# Autodesk Inventor assembly: BBM Staging Plate Assembly
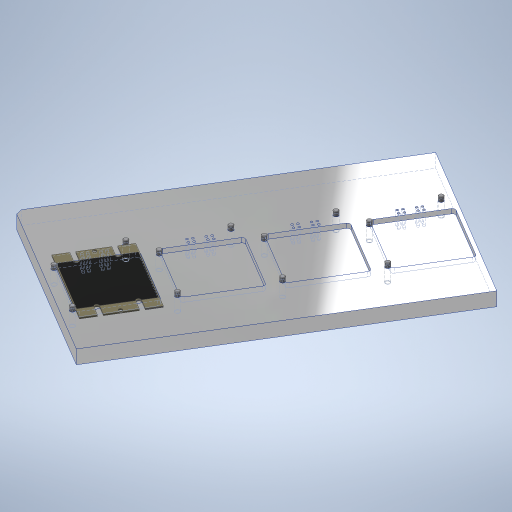
[picture p0: Inventor's stored thumbnail of the model, 512x512]
Saved by Autodesk Inventor 2023 (Build 270158000, 158)
## iProperties
Created: 2021-01-11
Part Number: BBM Staging Plate Assembly
Document SubType Name: Assembly
Designer: caleb
Author: caleb
## Documents named in this file (5)
- C:\Users\Caleb\Desktop\nebraska-silicon-lab\Hardware\ETL\Module Assembly\Baseplate Staging Plate - V2\Baseplate Staging Plate Assembly - V2.iam
- C:\Users\Caleb\Desktop\nebraska-silicon-lab\Hardware\ETL\Module Assembly\Baseplate Staging Plate - V2\Baseplate Staging Plate - V2.ipt
- C:\Users\Caleb\Desktop\nebraska-silicon-lab\Hardware\ETL\Module Assembly\Baseplate Staging Plate - V2\98381A304_Dowel Pin.ipt
- C:\Users\Caleb\Desktop\nebraska-silicon-lab\Hardware\ETL\modules\tamale v1.4\Coverplate Film.ipt
- C:\Users\Caleb\Desktop\nebraska-silicon-lab\Hardware\ETL\modules\tamale v1.4\Baseplate v1.4.ipt
## Components (15 placed, 4 different names)
1. Baseplate Staging Plate - V2:1 — Insert:1, Insert:2, Insert:3, Insert:4, Insert:5, Insert:6, Insert:7, Insert:8, Insert:9, Insert:10, Insert:11, Insert:12, Mate:6, Angle:1
2. 98381A304_Dowel Pin:1 — Insert:3, Tangent:1
3. 98381A304_Dowel Pin:2 — Insert:1, Tangent:2
4. 98381A304_Dowel Pin:3 — Insert:2
5. 98381A304_Dowel Pin:4 — Insert:4
6. 98381A304_Dowel Pin:5 — Insert:5
7. 98381A304_Dowel Pin:6 — Insert:6
8. 98381A304_Dowel Pin:7 — Insert:7
9. 98381A304_Dowel Pin:8 — Insert:8
10. 98381A304_Dowel Pin:9 — Insert:9
11. 98381A304_Dowel Pin:10 — Insert:10
12. 98381A304_Dowel Pin:11 — Insert:11
13. 98381A304_Dowel Pin:12 — Insert:12
14. Coverplate Film:1 — Flush:1, Flush:2
15. Baseplate v1.4:1 — Mate:6, Flush:1, Flush:2, Angle:1, Tangent:1, Tangent:2
## Relationships (19: Insert 12, Mate 2, Flush 2, Tangent 2, Angle 1)
- Insert:1: Baseplate Staging Plate - V2:1 ↔ 98381A304_Dowel Pin:2
- Insert:2: Baseplate Staging Plate - V2:1 ↔ 98381A304_Dowel Pin:3
- Insert:3: Baseplate Staging Plate - V2:1 ↔ 98381A304_Dowel Pin:1
- Insert:4: Baseplate Staging Plate - V2:1 ↔ 98381A304_Dowel Pin:4
- Insert:5: Baseplate Staging Plate - V2:1 ↔ 98381A304_Dowel Pin:5
- Insert:6: Baseplate Staging Plate - V2:1 ↔ 98381A304_Dowel Pin:6
- Insert:7: Baseplate Staging Plate - V2:1 ↔ 98381A304_Dowel Pin:7
- Insert:8: Baseplate Staging Plate - V2:1 ↔ 98381A304_Dowel Pin:8
- Insert:9: Baseplate Staging Plate - V2:1 ↔ 98381A304_Dowel Pin:9
- Insert:10: Baseplate Staging Plate - V2:1 ↔ 98381A304_Dowel Pin:10
- Insert:11: Baseplate Staging Plate - V2:1 ↔ 98381A304_Dowel Pin:11
- Insert:12: Baseplate Staging Plate - V2:1 ↔ 98381A304_Dowel Pin:12
- [Mate]: Coverplate Film:1 ↔ Baseplate v1.4:1
- Mate:6: Baseplate Staging Plate - V2:1 ↔ Baseplate v1.4:1
- Flush:1 (-0.55 mm): Coverplate Film:1 ↔ Baseplate v1.4:1
- Flush:2 (7.95 mm): Coverplate Film:1 ↔ Baseplate v1.4:1
- Angle:1 (0 deg): Baseplate Staging Plate - V2:1 ↔ Baseplate v1.4:1
- Tangent:1: 98381A304_Dowel Pin:1 ↔ Baseplate v1.4:1
- Tangent:2: 98381A304_Dowel Pin:2 ↔ Baseplate v1.4:1
